# Autodesk Inventor assembly: FrontLink
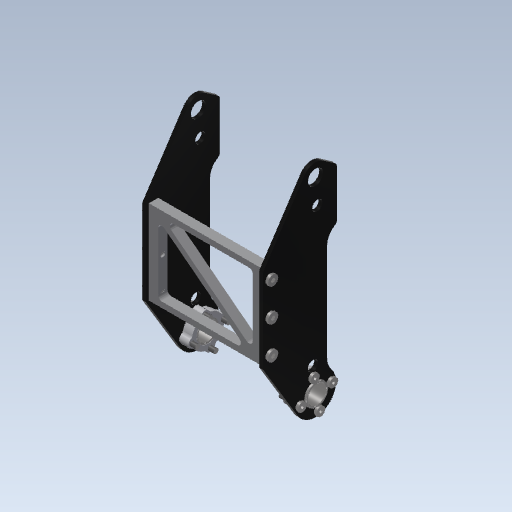
[picture p0: Inventor's stored thumbnail of the model, 512x512]
Saved by Autodesk Inventor 2020.4 (Build 244396000, 396)
## iProperties
Created: 2016-08-23
Part Number: FrontLink
Material: 一般
Document SubType Name: Assembly
Designer: hiro
Mass: 33.5175 g
Surface Area: 182.778 cm^2
Volume: 15.549 cm^3
Density: 2.15561 g/cm^3
Author: hiro
## Documents named in this file (7)
- C:\Users\Masato\Documents\Inventor\CIT Brains_Inventor\OpenPlatform_ver3_0\LowerBody\Link\FrontLink.iam
- C:\Users\Masato\Documents\Inventor\CIT Brains_Inventor\OpenPlatform_ver3_0\LowerBody\Link\FrontLink_diagonal.ipt
- C:\Users\Masato\Documents\Inventor\CIT Brains_Inventor\OpenPlatform_ver3_0\ReadyMade\Screw\M3-6.ipt
- C:\Users\Masato\Documents\Inventor\CIT Brains_Inventor\OpenPlatform_ver3_0\LowerBody\Link\FrontLink_frame.ipt
- C:\Users\Masato\Documents\Inventor\CIT Brains_Inventor\OpenPlatform_ver3_0\ReadyMade\Screw\M2_6-10.ipt
- C:\Users\Masato\Documents\Inventor\CIT Brains_Inventor\OpenPlatform_ver3_0\LowerBody\Knee\Knee_clamp.ipt
- C:\Users\Masato\Documents\Inventor\CIT Brains_Inventor\OpenPlatform_ver3_0\ReadyMade\Washer\WSSS-12-10-8.ipt
## Components (21 placed, 6 different names)
1. FrontLink_diagonal:1 — 挿入:1, 挿入:2, 挿入:3, 挿入:4, 挿入:5, 挿入:6, フラッシュ:1, メイト:1, メイト:2
2. FrontLink_frame:1 — 挿入:1, 挿入:2, 挿入:3, 挿入:7, 挿入:8, 挿入:9, 挿入:25, 挿入:27, 挿入:26, 挿入:28, 挿入:17, 挿入:18, 挿入:19, 挿入:20
3. FrontLink_frame:2 — 挿入:4, 挿入:5, 挿入:6, 挿入:10, 挿入:11, 挿入:12, 挿入:21, 挿入:22, 挿入:23, 挿入:24, 挿入:31, 挿入:29, 挿入:32, 挿入:30
4. Knee_clamp:1 — 挿入:15, 挿入:17, 挿入:18, 挿入:19, 挿入:20
5. Knee_clamp:2 — 挿入:16, 挿入:21, 挿入:22, 挿入:23, 挿入:24
6. WSSS-12-10-8:1 — 挿入:15
7. WSSS-12-10-8:2 — 挿入:16
8. M3-6:1 — 挿入:7
9. M3-6:2 — 挿入:8
10. M3-6:3 — 挿入:9
11. M3-6:4 — 挿入:10
12. M3-6:5 — 挿入:11
13. M3-6:6 — 挿入:12
14. M2_6-10:1 — 挿入:25
15. M2_6-10:2 — 挿入:26
16. M2_6-10:3 — 挿入:27
17. M2_6-10:4 — 挿入:28
18. M2_6-10:5 — 挿入:29
19. M2_6-10:6 — 挿入:30
20. M2_6-10:7 — 挿入:31
21. M2_6-10:8 — 挿入:32
## Relationships (33: Insert 30, Mate 2, Flush 1)
- 挿入:1 [Insert]: FrontLink_diagonal:1 ↔ FrontLink_frame:1
- 挿入:2 [Insert]: FrontLink_diagonal:1 ↔ FrontLink_frame:1
- 挿入:3 [Insert]: FrontLink_diagonal:1 ↔ FrontLink_frame:1
- 挿入:7 [Insert]: FrontLink_frame:1 ↔ M3-6:1
- 挿入:8 [Insert]: FrontLink_frame:1 ↔ M3-6:2
- 挿入:9 [Insert]: FrontLink_frame:1 ↔ M3-6:3
- 挿入:4 [Insert]: FrontLink_diagonal:1 ↔ FrontLink_frame:2
- 挿入:5 [Insert]: FrontLink_diagonal:1 ↔ FrontLink_frame:2
- 挿入:6 [Insert]: FrontLink_diagonal:1 ↔ FrontLink_frame:2
- 挿入:10 [Insert]: FrontLink_frame:2 ↔ M3-6:4
- 挿入:11 [Insert]: FrontLink_frame:2 ↔ M3-6:5
- 挿入:12 [Insert]: FrontLink_frame:2 ↔ M3-6:6
- 挿入:15 [Insert]: Knee_clamp:1 ↔ WSSS-12-10-8:1
- 挿入:16 [Insert]: Knee_clamp:2 ↔ WSSS-12-10-8:2
- 挿入:17 [Insert]: FrontLink_frame:1 ↔ Knee_clamp:1
- 挿入:18 [Insert]: FrontLink_frame:1 ↔ Knee_clamp:1
- 挿入:19 [Insert]: FrontLink_frame:1 ↔ Knee_clamp:1
- 挿入:20 [Insert]: FrontLink_frame:1 ↔ Knee_clamp:1
- 挿入:21 [Insert]: FrontLink_frame:2 ↔ Knee_clamp:2
- 挿入:22 [Insert]: FrontLink_frame:2 ↔ Knee_clamp:2
- 挿入:23 [Insert]: FrontLink_frame:2 ↔ Knee_clamp:2
- 挿入:24 [Insert]: FrontLink_frame:2 ↔ Knee_clamp:2
- 挿入:31 [Insert]: FrontLink_frame:2 ↔ M2_6-10:7
- 挿入:29 [Insert]: FrontLink_frame:2 ↔ M2_6-10:5
- 挿入:32 [Insert]: FrontLink_frame:2 ↔ M2_6-10:8
- 挿入:30 [Insert]: FrontLink_frame:2 ↔ M2_6-10:6
- 挿入:25 [Insert]: FrontLink_frame:1 ↔ M2_6-10:1
- 挿入:27 [Insert]: FrontLink_frame:1 ↔ M2_6-10:3
- 挿入:26 [Insert]: FrontLink_frame:1 ↔ M2_6-10:2
- 挿入:28 [Insert]: FrontLink_frame:1 ↔ M2_6-10:4
- フラッシュ:1 [Flush]: FrontLink_diagonal:1
- メイト:1 [Mate]: FrontLink_diagonal:1
- メイト:2 [Mate]: FrontLink_diagonal:1
